# Autodesk Inventor assembly: bearing
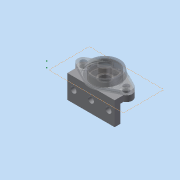
[picture p0: Inventor's stored thumbnail of the model, 180x180]
Saved by Autodesk Inventor 2015 (Build 190159000, 159)
## iProperties
Created: 2016-09-08
Part Number: bearing
Document SubType Name: Assembly
Designer: Dustin
Author: Dustin
## Documents named in this file (3)
- E:\Documents\3D Printer\Parts\New Printer\bearing.iam
- E:\Documents\3D Printer\Parts\New Printer\KFL08.iam
- E:\Documents\3D Printer\Parts\New Printer\leadscrew corners.ipt
## Components (2 placed, 2 different names)
1. KFL08:1 [sub-assembly] — Flush:1, Tangent:1
2. leadscrew corners:1 — Flush:1, Tangent:1
## Relationships (2: Flush 1, Tangent 1)
- Flush:1: KFL08:1 ↔ leadscrew corners:1
- Tangent:1: KFL08:1 ↔ leadscrew corners:1
